# Autodesk Inventor assembly: I.A.B 2.1 Aracet
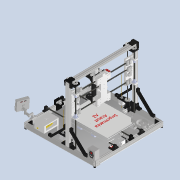
[picture p0: Inventor's stored thumbnail of the model, 180x180]
Saved by Autodesk Inventor 2020 (Build 240168000, 168)
## iProperties
Created: 2021-02-20
Part Number: I.A.B 2.1 Aracet
Document SubType Name: Assembly
Designer: Iulian Bors
Author: Iulian Bors
## Documents named in this file (72)
- Z:\I.A.B\Proiecte\0008 I.A.B 3D 2.1 Imprimanta aracet Metal\I.A.B 2.1 Aracet.iam
- Z:\I.A.B\Proiecte\0008 I.A.B 3D 2.1 Imprimanta aracet Metal\10 Mecanic\Foaie A3.ipt
- Z:\I.A.B\Proiecte\0008 I.A.B 3D 2.1 Imprimanta aracet Metal\10 Mecanic\0008-10-10 Injectomat Standard.iam
- Z:\I.A.B\Proiecte\0008 I.A.B 3D 2.1 Imprimanta aracet Metal\10 Mecanic\0008-10-006 suport injectomat.ipt
- Z:\I.A.B\Proiecte\0008 I.A.B 3D 2.1 Imprimanta aracet Metal\10 Mecanic\0008-10-1009 LM10uu.ipt
- Z:\I.A.B\Proiecte\0008 I.A.B 3D 2.1 Imprimanta aracet Metal\10 Mecanic\0008-10-007 Contra suport injectomat.ipt
- Z:\I.A.B\Proiecte\0008 I.A.B 3D 2.1 Imprimanta aracet Metal\10 Mecanic\0008-10-008 X Axis suport.ipt
- Z:\I.A.B\Proiecte\0008 I.A.B 3D 2.1 Imprimanta aracet Metal\10 Mecanic\0008-10-1001 NEMA17 - Motor de passo.ipt
- Z:\I.A.B\Proiecte\0008 I.A.B 3D 2.1 Imprimanta aracet Metal\10 Mecanic\0008-10-1011 GT2 Timing Pulley 20 Tooth.ipt
- Z:\I.A.B\Proiecte\0008 I.A.B 3D 2.1 Imprimanta aracet Metal\10 Mecanic\0008-10-009 X Axis suport.ipt
- Z:\I.A.B\Proiecte\0008 I.A.B 3D 2.1 Imprimanta aracet Metal\10 Mecanic\0008-10-010 Fixare AxaX.ipt
- Z:\I.A.B\Proiecte\0008 I.A.B 3D 2.1 Imprimanta aracet Metal\10 Mecanic\0008-10-011 Fixare AxaX Mijloc.ipt
- Z:\I.A.B\Proiecte\0008 I.A.B 3D 2.1 Imprimanta aracet Metal\10 Mecanic\0008-10-012 Intinzator X.ipt
- Z:\I.A.B\Proiecte\0008 I.A.B 3D 2.1 Imprimanta aracet Metal\10 Mecanic\0008-10-1012 16T W6 B3 Without T_Shrinkwrap_1.ipt
- Z:\I.A.B\Proiecte\0008 I.A.B 3D 2.1 Imprimanta aracet Metal\10 Mecanic\0008-10-1013 LMK 10 Bearing.ipt
- Z:\I.A.B\Proiecte\0008 I.A.B 3D 2.1 Imprimanta aracet Metal\10 Mecanic\0008-10-1010 Bara 10.ipt
- Z:\I.A.B\Proiecte\0008 I.A.B 3D 2.1 Imprimanta aracet Metal\10 Mecanic\0008-10-013 Supăort Piulita Axa Z.ipt
- Z:\I.A.B\Proiecte\0008 I.A.B 3D 2.1 Imprimanta aracet Metal\10 Mecanic\0008-10-1004 Piulita.ipt
- Z:\I.A.B\Proiecte\0008 I.A.B 3D 2.1 Imprimanta aracet Metal\10 Mecanic\0008-10-1014 T8 screw.ipt
- Z:\I.A.B\Proiecte\0008 I.A.B 3D 2.1 Imprimanta aracet Metal\10 Mecanic\0008-10-016 Suport Motor Z.ipt
- Z:\I.A.B\Proiecte\0008 I.A.B 3D 2.1 Imprimanta aracet Metal\10 Mecanic\0008-10-1005 ISO 1224-1 - 10 - 8 x 22 x 7.ipt
- Z:\I.A.B\Proiecte\0008 I.A.B 3D 2.1 Imprimanta aracet Metal\10 Mecanic\0008-10-015 roata condusa GT2.ipt
- Z:\I.A.B\Proiecte\0008 I.A.B 3D 2.1 Imprimanta aracet Metal\10 Mecanic\0008-10-1015 Synchronous Belt2.ipt
- Z:\I.A.B\Proiecte\0008 I.A.B 3D 2.1 Imprimanta aracet Metal\10 Mecanic\0008-10-017 Heated bed.ipt
- Z:\I.A.B\Proiecte\0008 I.A.B 3D 2.1 Imprimanta aracet Metal\10 Mecanic\0008-10-018 Suport Heated Bed.ipt
- Z:\I.A.B\Proiecte\0008 I.A.B 3D 2.1 Imprimanta aracet Metal\10 Mecanic\0008-10-1016 SC10UU.ipt
- Z:\I.A.B\Proiecte\0008 I.A.B 3D 2.1 Imprimanta aracet Metal\10 Mecanic\0008-10-1017 Bara 10.ipt
- Z:\I.A.B\Proiecte\0008 I.A.B 3D 2.1 Imprimanta aracet Metal\10 Mecanic\0008-10-019 Suport Axa Y.ipt
- Z:\I.A.B\Proiecte\0008 I.A.B 3D 2.1 Imprimanta aracet Metal\10 Mecanic\0008-10-1008 Bara 10_V1.ipt
- Z:\I.A.B\Proiecte\0008 I.A.B 3D 2.1 Imprimanta aracet Metal\10 Mecanic\0008-10-020 Suport Axa Y.ipt
- Z:\I.A.B\Proiecte\0008 I.A.B 3D 2.1 Imprimanta aracet Metal\10 Mecanic\0008-10-1018 V slot profiles.ipt
- Z:\I.A.B\Proiecte\0008 I.A.B 3D 2.1 Imprimanta aracet Metal\10 Mecanic\0008-10-1019 V slot profiles.ipt
- Z:\I.A.B\Proiecte\0008 I.A.B 3D 2.1 Imprimanta aracet Metal\10 Mecanic\0008-10-1020 V slot profiles.ipt
- Z:\I.A.B\Proiecte\0008 I.A.B 3D 2.1 Imprimanta aracet Metal\20 Electric\00008-20-1004 PowerSupplyLedMax500.ipt
- Z:\I.A.B\Proiecte\0008 I.A.B 3D 2.1 Imprimanta aracet Metal\10 Mecanic\0008-10-021 Suport Motor Z R.ipt
- Z:\I.A.B\Proiecte\0008 I.A.B 3D 2.1 Imprimanta aracet Metal\10 Mecanic\0008-10-1021  V slot profiles.ipt
- Z:\I.A.B\Proiecte\0008 I.A.B 3D 2.1 Imprimanta aracet Metal\10 Mecanic\0008-10-022 Tabla suport.ipt
- Z:\I.A.B\Proiecte\0008 I.A.B 3D 2.1 Imprimanta aracet Metal\10 Mecanic\0008-10-023 Suport L.ipt
- Z:\I.A.B\Proiecte\0008 I.A.B 3D 2.1 Imprimanta aracet Metal\10 Mecanic\0008-10-024 Ranforsare.ipt
- Z:\I.A.B\Proiecte\0008 I.A.B 3D 2.1 Imprimanta aracet Metal\10 Mecanic\0008-10-027 Cutie Arduino.ipt
- Z:\I.A.B\Proiecte\0008 I.A.B 3D 2.1 Imprimanta aracet Metal\10 Mecanic\0008-10-028 Cutie Elemente incalzire.ipt
- Z:\I.A.B\Proiecte\0008 I.A.B 3D 2.1 Imprimanta aracet Metal\20 Electric\0008-20-01 Assembly Arduino Mega RAMPS 1.4.iam
- Z:\I.A.B\Proiecte\0008 I.A.B 3D 2.1 Imprimanta aracet Metal\20 Electric\0008-20-1005 MOSFET_Step.ipt
- Z:\I.A.B\Proiecte\0008 I.A.B 3D 2.1 Imprimanta aracet Metal\10 Mecanic\0008-10-030 Suport L.ipt
- Z:\I.A.B\Proiecte\0008 I.A.B 3D 2.1 Imprimanta aracet Metal\10 Mecanic\0008-10-031 Suport L + placa.ipt
- Z:\I.A.B\Proiecte\0008 I.A.B 3D 2.1 Imprimanta aracet Metal\10 Mecanic\0008-10-1022 SHF10.ipt
- Z:\I.A.B\Proiecte\0008 I.A.B 3D 2.1 Imprimanta aracet Metal\10 Mecanic\0008-10-032 Suport cadru si axa Z.ipt
- Z:\I.A.B\Proiecte\0008 I.A.B 3D 2.1 Imprimanta aracet Metal\10 Mecanic\0008-10-033.ipt
- Z:\I.A.B\Proiecte\0008 I.A.B 3D 2.1 Imprimanta aracet Metal\10 Mecanic\0008-10-034 Suport_Rulment.ipt
- Z:\I.A.B\Proiecte\0008 I.A.B 3D 2.1 Imprimanta aracet Metal\10 Mecanic\0008-10-035.ipt
- Z:\I.A.B\Proiecte\0008 I.A.B 3D 2.1 Imprimanta aracet Metal\10 Mecanic\0008-10-037.ipt
- Z:\I.A.B\Proiecte\0008 I.A.B 3D 2.1 Imprimanta aracet Metal\10 Mecanic\0008-10-036.ipt
- Z:\I.A.B\Proiecte\0008 I.A.B 3D 2.1 Imprimanta aracet Metal\10 Mecanic\0008-10-11 ansamblu display.iam
- Z:\I.A.B\Proiecte\0008 I.A.B 3D 2.1 Imprimanta aracet Metal\10 Mecanic\0008-10-045.ipt
- Z:\I.A.B\Proiecte\0008 I.A.B 3D 2.1 Imprimanta aracet Metal\10 Mecanic\0008-10-044.ipt
- Z:\I.A.B\Proiecte\0008 I.A.B 3D 2.1 Imprimanta aracet Metal\10 Mecanic\0008-10-043.ipt
- Z:\I.A.B\Proiecte\0008 I.A.B 3D 2.1 Imprimanta aracet Metal\20 Electric\0008-20-1003 Switch.ipt
- Z:\I.A.B\Proiecte\0008 I.A.B 3D 2.1 Imprimanta aracet Metal\10 Mecanic\0008-10-046 Fixare axa si port cablu.ipt
- Z:\I.A.B\Proiecte\0008 I.A.B 3D 2.1 Imprimanta aracet Metal\10 Mecanic\0008-10-047 Suport Rulment Sc si curea.ipt
- Z:\I.A.B\Proiecte\0008 I.A.B 3D 2.1 Imprimanta aracet Metal\10 Mecanic\0008-10-048.ipt
- Z:\I.A.B\Proiecte\0008 I.A.B 3D 2.1 Imprimanta aracet Metal\10 Mecanic\0008-10-029 Capac Arduino.ipt
- Z:\I.A.B\Proiecte\0008 I.A.B 3D 2.1 Imprimanta aracet Metal\10 Mecanic\0008-10-049 Capac Mofset.ipt
- Z:\I.A.B\Proiecte\0008 I.A.B 3D 2.1 Imprimanta aracet Metal\10 Mecanic\Ansamblu nconector priza.iam
- Z:\I.A.B\Proiecte\0008 I.A.B 3D 2.1 Imprimanta aracet Metal\10 Mecanic\0008-10-056.ipt
- Z:\I.A.B\Proiecte\0008 I.A.B 3D 2.1 Imprimanta aracet Metal\10 Mecanic\0008-10-052 Suport Axa Y +Senzor.ipt
- Z:\I.A.B\Proiecte\0008 I.A.B 3D 2.1 Imprimanta aracet Metal\10 Mecanic\0008-10-026 Suport cutie.ipt
- Z:\I.A.B\Proiecte\0008 I.A.B 3D 2.1 Imprimanta aracet Metal\10 Mecanic\0008-10-053 picior.ipt
- Z:\I.A.B\Proiecte\0008 I.A.B 3D 2.1 Imprimanta aracet Metal\10 Mecanic\0008-10-054 Suport doking.ipt
- Z:\I.A.B\Proiecte\0008 I.A.B 3D 2.1 Imprimanta aracet Metal\10 Mecanic\0008-10-2016 DIN 315 - M4.ipt
- Z:\I.A.B\Proiecte\0008 I.A.B 3D 2.1 Imprimanta aracet Metal\10 Mecanic\0008-10-2017 DIN 7991 - M4x20.ipt
- Z:\I.A.B\Proiecte\0008 I.A.B 3D 2.1 Imprimanta aracet Metal\10 Mecanic\0008-10-055 Doking.ipt
- Z:\I.A.B\Proiecte\0008 I.A.B 3D 2.1 Imprimanta aracet Metal\10 Mecanic\0008-10-2000 DIN 6912 - M4 x 25.ipt
## Components (142 placed, 76 different names)
1. Foaie A3.ipt:1 — Mate:59, Flush:56, Flush:57, Angle:8, Mate:93
2. 0008-10-10 Injectomat Standard.iam:2 [sub-assembly] — Insert:10, Mate:64
3. 0008-10-006 suport injectomat.ipt:3 — Flush:3, Flush:4, Mate:8, Mate:9, Flush:5, Flush:6, Angle:2, Mate:17, Mate:23, Insert:10
4. 0008-10-1009 LM10uu.ipt:4 — Flush:1, Mate:5, Mate:8
5. 0008-10-1009 LM10uu.ipt:5 — Mate:5, Flush:121
6. 0008-10-1009 LM10uu.ipt:6 — Flush:4, Mate:6, Mate:9, Flush:1
7. 0008-10-1009 LM10uu.ipt:7 — Flush:3, Mate:6
8. 0008-10-007 Contra suport injectomat.ipt:8 — Flush:5, Flush:6, Mate:23, Mate:64, Flush:121, Flush:122, Mate:187, Flush:125, Flush:126
9. 0008-10-1008 Bara 10_V1.ipt:9
10. 0008-10-1008 Bara 10_V1.ipt:10 — Mate:188, Mate:189, Mate:191, Mate:192
11. 0008-10-009 X Axis suport.ipt:11 — Angle:2, Flush:10, Mate:21, Mate:22, Angle:3, Flush:26, Flush:27, Angle:4, Angle:5, Mate:26, Mate:27, Flush:32, Flush:34, Mate:38, Flush:36, Flush:37, Mate:163, Mate:164, Angle:28, Flush:127
12. 0008-10-008 X Axis suport.ipt:12 — Flush:10, Mate:21, Flush:31, Mate:30, Mate:31, Mate:33, Mate:34, Mate:35, Flush:89, Insert:21, Mate:172, Angle:25, Angle:29, Flush:128
13. 0008-10-1001 NEMA17 - Motor de passo.ipt:13 — Insert:1, Mate:22, Mate:26, Mate:27
14. 0008-10-1009 LM10uu.ipt:14 — Mate:17, Flush:122
15. 0008-10-1008 Bara 10_V1.ipt:15
16. 0008-10-1011 GT2 Timing Pulley 20 Tooth.ipt:16 — Insert:1, Flush:29, Flush:30, Angle:5
17. 0008-10-012 Intinzator X.ipt:17 — Flush:29, Insert:2, Flush:31
18. 0008-10-1012 16T W6 B3 Without T_Shrinkwrap_1.ipt:18 — Insert:2, Flush:30
19. 0008-10-1013 LMK 10 Bearing.ipt:19 — Mate:29, Angle:6, Mate:164
20. 0008-10-1013 LMK 10 Bearing.ipt:20 — Mate:33, Mate:34, Mate:35
21. 0008-10-1013 LMK 10 Bearing.ipt:21 — Mate:30, Mate:31, Mate:37, Angle:25
22. 0008-10-1013 LMK 10 Bearing.ipt:22 — Flush:32, Mate:29, Flush:34, Angle:6, Mate:36
23. 0008-10-010 Fixare AxaX.ipt:23 — Angle:3, Flush:26
24. 0008-10-1010 Bara 10.ipt:31 — Mate:36, Flush:35, Insert:15, Insert:16, Mate:163
25. 0008-10-1010 Bara 10.ipt:32 — Mate:37, Flush:35, Insert:17, Insert:18
26. 0008-10-013 Supăort Piulita Axa Z.ipt:33 — Mate:38, Flush:36, Mate:39, Mate:40, Flush:37, Flush:38
27. 0008-10-1004 Piulita.ipt:34 — Mate:39, Mate:40, Flush:38, Mate:44
28. 0008-10-013 Supăort Piulita Axa Z.ipt:35 — Insert:21, Mate:172, Mate:173, Mate:174
29. 0008-10-1004 Piulita.ipt:36 — Mate:45, Mate:173, Mate:174
30. 0008-10-1014 T8 screw.ipt:37 — Mate:44, Mate:47, Mate:50, Mate:168
31. 0008-10-1014 T8 screw.ipt:38 — Mate:45, Mate:57, Mate:58, Mate:82, Mate:113, Mate:171, Mate:176
32. 0008-10-016 Suport Motor Z.ipt:39 — Mate:47, Mate:48, Mate:49, Insert:6, Mate:101, Mate:103, Mate:104, Angle:14
33. 0008-10-1005 ISO 1224-1 - 10 - 8 x 22 x 7.ipt:40 — Insert:4, Insert:6
34. 0008-10-015 roata condusa GT2.ipt:41 — Insert:4, Mate:202
35. 0008-10-1001 NEMA17 - Motor de passo.ipt:42 — Insert:5, Mate:48, Mate:49
36. 0008-10-1011 GT2 Timing Pulley 20 Tooth.ipt:43 — Insert:5, Mate:51, Mate:52
37. 0008-10-1015 Synchronous Belt2.ipt:44 — Mate:50, Mate:51, Mate:52, Mate:202
38. 0008-10-016 Suport Motor Z.ipt:45 — Mate:82, Mate:87, Angle:15, Mate:107
39. 0008-10-1005 ISO 1224-1 - 10 - 8 x 22 x 7.ipt:46
40. 0008-10-015 roata condusa GT2.ipt:47 — Mate:57
41. 0008-10-1001 NEMA17 - Motor de passo.ipt:48 — Angle:16, Mate:113
42. 0008-10-1011 GT2 Timing Pulley 20 Tooth.ipt:49
43. 0008-10-1015 Synchronous Belt2.ipt:50 — Mate:58
44. 0008-10-017 Heated bed.ipt:51 — Mate:59, Flush:56, Flush:57, Mate:60, Mate:61, Mate:62
45. 0008-10-018 Suport Heated Bed.ipt:52 — Mate:60, Mate:61, Mate:62, Mate:65, Flush:59, Mate:66, Flush:61, Mate:68, Mate:69, Flush:64, Flush:65, Angle:9, Mate:73, Mate:74, Mate:78, Mate:197, Insert:32, Mate:210, Insert:33, Insert:36, Angle:32
46. 0008-10-1016 SC10UU.ipt:55 — Mate:69, Flush:63, Flush:64
47. 0008-10-1016 SC10UU.ipt:56 — Mate:66, Mate:67, Flush:60, Flush:63
48. 0008-10-1016 SC10UU.ipt:57 — Mate:68, Flush:62, Flush:65, Mate:70
49. 0008-10-1016 SC10UU.ipt:58 — Mate:65, Flush:59, Mate:67, Flush:60, Flush:61, Flush:62, Mate:77
50. 0008-10-1017 Bara 10.ipt:59 — Mate:70, Mate:71, Flush:66, Flush:67, Mate:72
51. 0008-10-019 Suport Axa Y.ipt:60 — Mate:71, Flush:66, Angle:9, Angle:10, Flush:70, Flush:71, Flush:73, Flush:74
52. 0008-10-019 Suport Axa Y.ipt:61 — Angle:10, Flush:67, Mate:72, Flush:75, Mate:208, Flush:138
53. 0008-10-1016 SC10UU:5 — Mate:73, Mate:74, Mate:78, Mate:79, Mate:198, Mate:199
54. 0008-10-1017 Bara 10:2 — Mate:77, Flush:72
55. 0008-10-020 Suport Axa Y:4 — Flush:70, Flush:71, Mate:135
56. 0008-10-020 Suport Axa Y:6 — Angle:12
57. 0008-10-1017 Bara 10:3 — Mate:79, Flush:72, Mate:80, Mate:81
58. 0008-10-019 Suport Axa Y:2 — Mate:80, Flush:73, Flush:74, Mate:83, Flush:77, Angle:27, Mate:182
59. 0008-10-019 Suport Axa Y:1 — Mate:81, Flush:75, Angle:12
60. 0008-10-1018 V slot profiles:1 — Mate:83, Flush:77, Flush:78, Mate:85, Flush:79, Flush:80, Mate:86, Flush:81, Mate:93, Mate:109, Flush:101, Mate:112, Mate:114, Angle:17, Mate:136, Flush:110, Mate:183, Mate:186, Flush:123, Flush:124
61. 0008-10-1019 V slot profiles:1 — Flush:78, Mate:85, Flush:79, Mate:100, Flush:96, Mate:101, Angle:14, Mate:105, Flush:102, Mate:111, Flush:104, Mate:122, Mate:123, Flush:105, Mate:125, Flush:106, Mate:129, Flush:108, Mate:152, Mate:156, Mate:157, Angle:20, Mate:205, Flush:133
62. 0008-10-1019 V slot profiles:2 — Flush:80, Mate:86, Flush:81, Mate:87, Flush:82, Flush:85, Mate:90, Flush:94, Mate:99, Flush:95, Angle:15, Mate:106, Flush:100, Angle:16, Mate:116, Mate:119, Mate:127, Mate:132, Mate:141, Flush:113, Mate:143, Flush:114, Mate:146, Mate:149, Angle:19
63. 0008-10-1018 V slot profiles:2 — Flush:82, Flush:85, Mate:90, Mate:97, Flush:99, Mate:108, Flush:103, Mate:118, Mate:121, Mate:200, Flush:131, Flush:134
64. 0008-10-1018 V slot profiles:3 — Flush:97, Flush:98, Mate:110, Mate:161, Angle:22, Mate:165, Flush:116, Angle:24, Mate:170, Mate:177
65. 0008-10-1020 V slot profiles:2 — Flush:89, Flush:91, Mate:99, Flush:95, Flush:97, Flush:98, Mate:128, Flush:107, Mate:131, Flush:109, Mate:142, Mate:144, Mate:169, Flush:117, Flush:118, Mate:178
66. 0008-10-1020 V slot profiles:3 — Flush:91, Mate:100, Flush:96, Flush:103, Mate:110, Mate:124, Mate:126, Mate:158, Mate:159, Mate:162, Flush:115, Mate:166, Mate:207, Flush:137
67. 0008-10-1001 NEMA17 - Motor de passo:4 — Mate:97, Flush:99, Mate:201
68. 0008-10-1011 GT2 Timing Pulley 20 Tooth:4 — Flush:120
69. 00008-20-1004 PowerSupplyLedMax500:1 — Flush:94, Mate:108, Flush:130, Mate:195, Mate:196
70. 0008-10-1021  V slot profiles:1 — Mate:103, Mate:104, Mate:105, Mate:153, Mate:155, Flush:132
71. 0008-10-1021  V slot profiles:2 — Mate:106, Mate:107, Flush:100, Mate:147, Mate:150, Flush:132
72. 0008-10-022 Tabla suport:1 — Mate:109, Flush:101, Flush:102, Mate:115, Mate:117, Mate:120, Mate:130, Mate:145, Mate:148, Mate:151, Mate:154, Mate:160, Mate:180, Mate:194, Insert:28, Insert:29, Insert:30, Insert:31
73. 0008-10-023 Suport L:1 — Mate:111, Flush:104, Mate:112
74. 0008-10-023 Suport L:2 — Mate:120, Mate:121, Mate:122
75. 0008-10-023 Suport L:3 — Mate:117, Mate:118, Mate:119, Mate:196
76. 0008-10-023 Suport L:4 — Mate:114, Mate:115, Mate:116
77. 0008-10-024 Ranforsare:1 — Mate:123, Flush:105, Mate:124
78. 0008-10-024 Ranforsare:2 — Mate:127, Mate:128, Flush:107
79. 0008-10-024 Ranforsare:3 — Mate:125, Mate:126, Flush:106
80. 0008-10-027 Cutie Arduino:1 — Mate:129, Flush:108, Insert:12, Angle:18, Flush:110, Insert:26, Angle:30, Insert:27, Mate:209
81. 0008-10-028 Cutie Elemente incalzire:1 — Mate:130, Angle:17, Insert:13, Mate:133, Insert:14, Mate:134, Mate:135, Mate:136, Mate:203, Mate:204, Angle:31
82. 0008-10-024 Ranforsare:4 — Mate:131, Flush:109, Mate:132
83. 0008-20-01 Assembly Arduino Mega RAMPS 1.4:1 [sub-assembly] — Insert:12, Angle:18
84. 0008-20-1005 MOSFET_Step:1 — Insert:13, Mate:133
85. 0008-20-1005 MOSFET_Step:2 — Insert:14, Mate:134
86. 0008-10-031 Suport L + placa:1 — Mate:143, Mate:144, Flush:114
87. 0008-10-030 Suport L:4 — Mate:141, Mate:142, Flush:113
88. 0008-10-030 Suport L:5 — Mate:145, Mate:146, Mate:147
89. 0008-10-030 Suport L:6 — Mate:148, Mate:149, Mate:150
90. 0008-10-031 Suport L + placa:2 — Mate:157, Mate:158, Mate:159
91. 0008-10-030 Suport L:7 — Mate:151, Mate:152, Mate:153
92. 0008-10-030 Suport L:8 — Mate:154, Mate:155, Mate:156
93. 0008-10-1022 SHF10:1 — Insert:16, Mate:160, Angle:20
94. 0008-10-1022 SHF10:2 — Insert:18, Angle:19
95. 0008-10-1022 SHF10:3 — Insert:17, Angle:22
96. 0008-10-1022 SHF10:4 — Insert:15, Angle:23
97. 0008-10-032 Suport cadru si axa Z:1 — Mate:161, Mate:162, Flush:115
98. 0008-10-033:1 — Mate:165, Flush:116, Mate:166, Angle:23, Mate:167
99. 0008-10-034 Suport_Rulment:1 — Mate:167, Angle:24
100. ISO 1224-1 (Metric) 10 - 8 x 16 x 7:3 — Mate:168
101. 0008-10-035:1 — Mate:169, Flush:117, Mate:170, Mate:171, Mate:175
102. 0008-10-034 Suport_Rulment:2 — Mate:175
103. ISO 1224-1 (Metric) 10 - 8 x 16 x 7:4 — Mate:176
104. 0008-10-032 Suport cadru si axa Z:2 — Mate:177, Flush:118, Mate:178
105. 0008-10-037:1 — Mate:180, Mate:181, Mate:182, Mate:183, Mate:184
106. 0008-10-036:1 — Insert:22, Angle:27, Mate:181, Mate:184
107. 0008-10-1012 16T W6 B3 Without T_Shrinkwrap_1:2 — Insert:22, Flush:120
108. 0008-10-11 ansamblu display:1 [sub-assembly] — Insert:23, Mate:185
109. 0008-10-045:1 — Insert:23, Mate:185, Insert:24
110. 0008-10-044:1 — Insert:24, Insert:25
111. 0008-10-043:1 — Mate:186, Flush:123, Insert:25, Flush:124
112. 0008-20-1003 Switch:1 — Mate:187, Flush:125, Flush:126
113. 0008-10-010 Fixare AxaX:2 — Mate:188, Angle:28, Flush:127, Mate:190
114. 0008-10-010 Fixare AxaX:4 — Mate:189, Mate:190
115. 00008-20-1004 PowerSupplyLedMax500:2 — Mate:194, Flush:130, Mate:195
116. 0008-10-047 Suport Rulment Sc si curea:1 — Mate:197, Mate:198, Mate:199
117. 0008-10-048:1 — Mate:200, Mate:201, Flush:131
118. 0008-10-029 Capac Arduino:1 — Insert:26, Angle:30
119. 0008-10-049 Capac Mofset:1 — Mate:203, Mate:204, Angle:31
120. Ansamblu nconector priza:1 [sub-assembly] — Mate:205, Flush:133, Flush:134
121. 0008-20-1003 Switch:2 — Mate:206, Flush:135, Flush:136
122. 0008-10-056:1 — Mate:206, Flush:135, Flush:136, Mate:207, Flush:137
123. 0008-20-1003 Switch:3 — Mate:208, Flush:138
124. 0008-10-026 Suport cutie:1 — Insert:27, Mate:209
125. 0008-10-053 picior:1 — Insert:28
126. 0008-10-053 picior:3 — Insert:31
127. 0008-10-053 picior:4 — Insert:30
128. 0008-10-053 picior:5 — Insert:29
129. 0008-10-054 Suport doking:1 — Insert:32, Mate:210, Flush:139, Mate:211, Mate:212, Insert:39
130. DIN 315 M4:1 — Insert:34
131. DIN 7991 M4x20:1 — Insert:33, Insert:34
132. DIN 315 M4:2
133. DIN 7991 M4x20:2 — Insert:36
134. 0008-10-055 Doking:1 — Flush:139, Angle:32, Mate:211, Mate:212
135. DIN 315 M4:3 — Insert:40
136. DIN 6912 M4 x 25:1 — Insert:39, Insert:40
137. 0008-10-011 Fixare AxaX Mijloc.ipt:53 — Flush:27, Angle:4
138. 0008-10-011 Fixare AxaX Mijloc.ipt:54
139. 0008-10-010 Fixare AxaX:5 — Mate:191, Angle:29, Flush:128, Flush:129, Mate:193
140. 0008-10-010 Fixare AxaX:3 — Mate:192, Flush:129, Mate:193
141. 0008-10-010 Fixare AxaX:6
142. 0008-10-010 Fixare AxaX:7
## Component patterns: (2 elements, first: 0008-10-011 Fixare AxaX Mijloc.ipt:53), (2 elements, first: 0008-10-010 Fixare AxaX:5 + 0008-10-010 Fixare AxaX:3)
## Relationships (336: Mate 179, Flush 92, Insert 37, Angle 27, Tangent 1)
- Flush:1 (20 mm): 0008-10-1009 LM10uu.ipt:4 ↔ 0008-10-1009 LM10uu.ipt:6
- Mate:5: 0008-10-1009 LM10uu.ipt:4 ↔ 0008-10-1009 LM10uu.ipt:5
- Flush:3 (20 mm): 0008-10-006 suport injectomat.ipt:3 ↔ 0008-10-1009 LM10uu.ipt:7
- Flush:4 (20 mm): 0008-10-006 suport injectomat.ipt:3 ↔ 0008-10-1009 LM10uu.ipt:6
- Mate:6: 0008-10-1009 LM10uu.ipt:6 ↔ 0008-10-1009 LM10uu.ipt:7
- Mate:8: 0008-10-006 suport injectomat.ipt:3 ↔ 0008-10-1009 LM10uu.ipt:4
- Mate:9: 0008-10-006 suport injectomat.ipt:3 ↔ 0008-10-1009 LM10uu.ipt:6
- Flush:5: 0008-10-006 suport injectomat.ipt:3 ↔ 0008-10-007 Contra suport injectomat.ipt:8
- Flush:6: 0008-10-006 suport injectomat.ipt:3 ↔ 0008-10-007 Contra suport injectomat.ipt:8
- [Mate]: 0008-10-1009 LM10uu.ipt:5 ↔ 0008-10-1008 Bara 10_V1.ipt:9
- [Mate]: 0008-10-1009 LM10uu.ipt:7 ↔ 0008-10-1008 Bara 10_V1.ipt:10
- [Flush]: 0008-10-1008 Bara 10_V1.ipt:9 ↔ 0008-10-1008 Bara 10_V1.ipt:10
- [Tangent] (-3 mm): 0008-10-1008 Bara 10_V1.ipt:9 ↔ 0008-10-009 X Axis suport.ipt:11
- Angle:2 (0 deg): 0008-10-006 suport injectomat.ipt:3 ↔ 0008-10-009 X Axis suport.ipt:11
- [Flush] (-30 mm): 0008-10-1008 Bara 10_V1.ipt:9 ↔ 0008-10-009 X Axis suport.ipt:11
- Flush:10: 0008-10-009 X Axis suport.ipt:11 ↔ 0008-10-008 X Axis suport.ipt:12
- [Flush] (-30 mm): 0008-10-1008 Bara 10_V1.ipt:9 ↔ 0008-10-008 X Axis suport.ipt:12
- Mate:21: 0008-10-009 X Axis suport.ipt:11 ↔ 0008-10-008 X Axis suport.ipt:12
- [Mate]: Foaie A3.ipt:1 ↔ 0008-10-1008 Bara 10_V1.ipt:9
- Mate:17: 0008-10-006 suport injectomat.ipt:3 ↔ 0008-10-1009 LM10uu.ipt:14
- Insert:1: 0008-10-1001 NEMA17 - Motor de passo.ipt:13 ↔ 0008-10-1011 GT2 Timing Pulley 20 Tooth.ipt:16
- Mate:22 (-10 mm): 0008-10-009 X Axis suport.ipt:11 ↔ 0008-10-1001 NEMA17 - Motor de passo.ipt:13
- Mate:23 (2 mm): 0008-10-006 suport injectomat.ipt:3 ↔ 0008-10-007 Contra suport injectomat.ipt:8
- [Flush]: 0008-10-1008 Bara 10_V1.ipt:9 ↔ 0008-10-1008 Bara 10_V1.ipt:15
- [Mate]: 0008-10-1009 LM10uu.ipt:14 ↔ 0008-10-1008 Bara 10_V1.ipt:15
- [Mate]: 0008-10-1008 Bara 10_V1.ipt:9 ↔ 0008-10-010 Fixare AxaX.ipt:23
- Angle:3 (0 deg): 0008-10-009 X Axis suport.ipt:11 ↔ 0008-10-010 Fixare AxaX.ipt:23
- Flush:26 (35 mm): 0008-10-009 X Axis suport.ipt:11 ↔ 0008-10-010 Fixare AxaX.ipt:23
- [Mate]: 0008-10-1008 Bara 10_V1.ipt:15 ↔ 0008-10-011 Fixare AxaX Mijloc.ipt:53
- Flush:27 (30 mm): 0008-10-009 X Axis suport.ipt:11 ↔ 0008-10-011 Fixare AxaX Mijloc.ipt:53
- Angle:4 (0 deg): 0008-10-009 X Axis suport.ipt:11 ↔ 0008-10-011 Fixare AxaX Mijloc.ipt:53
- Flush:29: 0008-10-1011 GT2 Timing Pulley 20 Tooth.ipt:16 ↔ 0008-10-012 Intinzator X.ipt:17
- Insert:2 (0.25 mm): 0008-10-012 Intinzator X.ipt:17 ↔ 0008-10-1012 16T W6 B3 Without T_Shrinkwrap_1.ipt:18
- Flush:30: 0008-10-1011 GT2 Timing Pulley 20 Tooth.ipt:16 ↔ 0008-10-1012 16T W6 B3 Without T_Shrinkwrap_1.ipt:18
- Flush:31: 0008-10-008 X Axis suport.ipt:12 ↔ 0008-10-012 Intinzator X.ipt:17
- Angle:5 (0 deg): 0008-10-009 X Axis suport.ipt:11 ↔ 0008-10-1011 GT2 Timing Pulley 20 Tooth.ipt:16
- Mate:26 (1 mm): 0008-10-009 X Axis suport.ipt:11 ↔ 0008-10-1001 NEMA17 - Motor de passo.ipt:13
- Mate:27 (1 mm): 0008-10-009 X Axis suport.ipt:11 ↔ 0008-10-1001 NEMA17 - Motor de passo.ipt:13
- Flush:32 (15 mm): 0008-10-009 X Axis suport.ipt:11 ↔ 0008-10-1013 LMK 10 Bearing.ipt:22
- Mate:29: 0008-10-1013 LMK 10 Bearing.ipt:19 ↔ 0008-10-1013 LMK 10 Bearing.ipt:22
- Flush:34: 0008-10-009 X Axis suport.ipt:11 ↔ 0008-10-1013 LMK 10 Bearing.ipt:22
- Angle:6 (0 deg): 0008-10-1013 LMK 10 Bearing.ipt:19 ↔ 0008-10-1013 LMK 10 Bearing.ipt:22
- Mate:30: 0008-10-008 X Axis suport.ipt:12 ↔ 0008-10-1013 LMK 10 Bearing.ipt:21
- Mate:31: 0008-10-008 X Axis suport.ipt:12 ↔ 0008-10-1013 LMK 10 Bearing.ipt:21
- Mate:33: 0008-10-008 X Axis suport.ipt:12 ↔ 0008-10-1013 LMK 10 Bearing.ipt:20
- Mate:34: 0008-10-008 X Axis suport.ipt:12 ↔ 0008-10-1013 LMK 10 Bearing.ipt:20
- Mate:35: 0008-10-008 X Axis suport.ipt:12 ↔ 0008-10-1013 LMK 10 Bearing.ipt:20
- Mate:36: 0008-10-1013 LMK 10 Bearing.ipt:22 ↔ 0008-10-1010 Bara 10.ipt:31
- Mate:37: 0008-10-1013 LMK 10 Bearing.ipt:21 ↔ 0008-10-1010 Bara 10.ipt:32
- Flush:35: 0008-10-1010 Bara 10.ipt:31 ↔ 0008-10-1010 Bara 10.ipt:32
- Mate:38: 0008-10-009 X Axis suport.ipt:11 ↔ 0008-10-013 Supăort Piulita Axa Z.ipt:33
- Flush:36: 0008-10-009 X Axis suport.ipt:11 ↔ 0008-10-013 Supăort Piulita Axa Z.ipt:33
- Mate:39: 0008-10-013 Supăort Piulita Axa Z.ipt:33 ↔ 0008-10-1004 Piulita.ipt:34
- Mate:40 (-12 mm): 0008-10-013 Supăort Piulita Axa Z.ipt:33 ↔ 0008-10-1004 Piulita.ipt:34
- Flush:37 (80 mm): 0008-10-009 X Axis suport.ipt:11 ↔ 0008-10-013 Supăort Piulita Axa Z.ipt:33
- Flush:38 (15 mm): 0008-10-013 Supăort Piulita Axa Z.ipt:33 ↔ 0008-10-1004 Piulita.ipt:34
- Mate:44: 0008-10-1004 Piulita.ipt:34 ↔ 0008-10-1014 T8 screw.ipt:37
- Mate:45: 0008-10-1004 Piulita.ipt:36 ↔ 0008-10-1014 T8 screw.ipt:38
- Insert:4: 0008-10-1005 ISO 1224-1 - 10 - 8 x 22 x 7.ipt:40 ↔ 0008-10-015 roata condusa GT2.ipt:41
- Mate:47 (1 mm): 0008-10-1014 T8 screw.ipt:37 ↔ 0008-10-016 Suport Motor Z.ipt:39
- Insert:5: 0008-10-1001 NEMA17 - Motor de passo.ipt:42 ↔ 0008-10-1011 GT2 Timing Pulley 20 Tooth.ipt:43
- Mate:48: 0008-10-016 Suport Motor Z.ipt:39 ↔ 0008-10-1001 NEMA17 - Motor de passo.ipt:42
- Mate:49: 0008-10-016 Suport Motor Z.ipt:39 ↔ 0008-10-1001 NEMA17 - Motor de passo.ipt:42
- Mate:50: 0008-10-1014 T8 screw.ipt:37 ↔ 0008-10-1015 Synchronous Belt2.ipt:44
- Mate:51: 0008-10-1011 GT2 Timing Pulley 20 Tooth.ipt:43 ↔ 0008-10-1015 Synchronous Belt2.ipt:44
- Mate:52 (1.5 mm): 0008-10-1011 GT2 Timing Pulley 20 Tooth.ipt:43 ↔ 0008-10-1015 Synchronous Belt2.ipt:44
- Insert:6: 0008-10-016 Suport Motor Z.ipt:39 ↔ 0008-10-1005 ISO 1224-1 - 10 - 8 x 22 x 7.ipt:40
- [Insert]: 0008-10-1005 ISO 1224-1 - 10 - 8 x 22 x 7.ipt:46 ↔ 0008-10-015 roata condusa GT2.ipt:47
- [Insert]: 0008-10-1001 NEMA17 - Motor de passo.ipt:48 ↔ 0008-10-1011 GT2 Timing Pulley 20 Tooth.ipt:49
- [Mate]: 0008-10-016 Suport Motor Z.ipt:45 ↔ 0008-10-1001 NEMA17 - Motor de passo.ipt:48
- [Mate]: 0008-10-1011 GT2 Timing Pulley 20 Tooth.ipt:49 ↔ 0008-10-1015 Synchronous Belt2.ipt:50
- [Mate] (1.5 mm): 0008-10-1011 GT2 Timing Pulley 20 Tooth.ipt:49 ↔ 0008-10-1015 Synchronous Belt2.ipt:50
- [Insert]: 0008-10-016 Suport Motor Z.ipt:45 ↔ 0008-10-1005 ISO 1224-1 - 10 - 8 x 22 x 7.ipt:46
- Mate:57: 0008-10-1014 T8 screw.ipt:38 ↔ 0008-10-015 roata condusa GT2.ipt:47
- Mate:58: 0008-10-1014 T8 screw.ipt:38 ↔ 0008-10-1015 Synchronous Belt2.ipt:50
- Mate:59: Foaie A3.ipt:1 ↔ 0008-10-017 Heated bed.ipt:51
- Flush:56 (-10 mm): Foaie A3.ipt:1 ↔ 0008-10-017 Heated bed.ipt:51
- Flush:57 (-10 mm): Foaie A3.ipt:1 ↔ 0008-10-017 Heated bed.ipt:51
- Mate:60 (25 mm): 0008-10-017 Heated bed.ipt:51 ↔ 0008-10-018 Suport Heated Bed.ipt:52
- Mate:61: 0008-10-017 Heated bed.ipt:51 ↔ 0008-10-018 Suport Heated Bed.ipt:52
- Mate:62: 0008-10-017 Heated bed.ipt:51 ↔ 0008-10-018 Suport Heated Bed.ipt:52
- Angle:8 (0 deg): Foaie A3.ipt:1
- [Mate]: 0008-10-1008 Bara 10_V1.ipt:9 ↔ 0008-10-009 X Axis suport.ipt:11
- Insert:10: 0008-10-10 Injectomat Standard.iam:2 ↔ 0008-10-006 suport injectomat.ipt:3
- Mate:64: 0008-10-10 Injectomat Standard.iam:2 ↔ 0008-10-007 Contra suport injectomat.ipt:8
- Mate:65: 0008-10-018 Suport Heated Bed.ipt:52 ↔ 0008-10-1016 SC10UU.ipt:58
- Flush:59 (5 mm): 0008-10-018 Suport Heated Bed.ipt:52 ↔ 0008-10-1016 SC10UU.ipt:58
- Mate:66: 0008-10-018 Suport Heated Bed.ipt:52 ↔ 0008-10-1016 SC10UU.ipt:56
- Mate:67 (100 mm): 0008-10-1016 SC10UU.ipt:56 ↔ 0008-10-1016 SC10UU.ipt:58
- Flush:60: 0008-10-1016 SC10UU.ipt:56 ↔ 0008-10-1016 SC10UU.ipt:58
- Flush:61 (135 mm): 0008-10-018 Suport Heated Bed.ipt:52 ↔ 0008-10-1016 SC10UU.ipt:58
- Mate:68: 0008-10-018 Suport Heated Bed.ipt:52 ↔ 0008-10-1016 SC10UU.ipt:57
- Flush:62: 0008-10-1016 SC10UU.ipt:57 ↔ 0008-10-1016 SC10UU.ipt:58
- Mate:69: 0008-10-018 Suport Heated Bed.ipt:52 ↔ 0008-10-1016 SC10UU.ipt:55
- Flush:63: 0008-10-1016 SC10UU.ipt:55 ↔ 0008-10-1016 SC10UU.ipt:56
- Flush:64 (5 mm): 0008-10-018 Suport Heated Bed.ipt:52 ↔ 0008-10-1016 SC10UU.ipt:55
- Flush:65 (5 mm): 0008-10-018 Suport Heated Bed.ipt:52 ↔ 0008-10-1016 SC10UU.ipt:57
- Mate:70: 0008-10-1016 SC10UU.ipt:57 ↔ 0008-10-1017 Bara 10.ipt:59
- Mate:71: 0008-10-1017 Bara 10.ipt:59 ↔ 0008-10-019 Suport Axa Y.ipt:60
- Flush:66: 0008-10-1017 Bara 10.ipt:59 ↔ 0008-10-019 Suport Axa Y.ipt:60
- Angle:9 (0 deg): 0008-10-018 Suport Heated Bed.ipt:52 ↔ 0008-10-019 Suport Axa Y.ipt:60
- Angle:10 (0 deg): 0008-10-019 Suport Axa Y.ipt:60 ↔ 0008-10-019 Suport Axa Y.ipt:61
- Flush:67: 0008-10-1017 Bara 10.ipt:59 ↔ 0008-10-019 Suport Axa Y.ipt:61
- Mate:72: 0008-10-1017 Bara 10.ipt:59 ↔ 0008-10-019 Suport Axa Y.ipt:61
- Mate:73 (5 mm): 0008-10-018 Suport Heated Bed.ipt:52 ↔ 0008-10-1016 SC10UU:5
- Mate:74 (30 mm): 0008-10-018 Suport Heated Bed.ipt:52 ↔ 0008-10-1016 SC10UU:5
- [Mate]: 0008-10-1017 Bara 10:2 ↔ 0008-10-020 Suport Axa Y:4
- [Flush]: 0008-10-1017 Bara 10:2 ↔ 0008-10-020 Suport Axa Y:4
- [Angle] (0 deg): 0008-10-020 Suport Axa Y:4 ↔ 0008-10-020 Suport Axa Y:6
- [Flush]: 0008-10-1017 Bara 10:2 ↔ 0008-10-020 Suport Axa Y:6
- [Mate]: 0008-10-1017 Bara 10:2 ↔ 0008-10-020 Suport Axa Y:6
- Mate:77: 0008-10-1016 SC10UU.ipt:58 ↔ 0008-10-1017 Bara 10:2
- Mate:78 (-17.5 mm): 0008-10-018 Suport Heated Bed.ipt:52 ↔ 0008-10-1016 SC10UU:5
- Flush:70: 0008-10-019 Suport Axa Y.ipt:60 ↔ 0008-10-020 Suport Axa Y:4
- Flush:71: 0008-10-019 Suport Axa Y.ipt:60 ↔ 0008-10-020 Suport Axa Y:4
- Mate:79: 0008-10-1016 SC10UU:5 ↔ 0008-10-1017 Bara 10:3
- Flush:72: 0008-10-1017 Bara 10:2 ↔ 0008-10-1017 Bara 10:3
- Mate:80: 0008-10-1017 Bara 10:3 ↔ 0008-10-019 Suport Axa Y:2
- Flush:73: 0008-10-019 Suport Axa Y.ipt:60 ↔ 0008-10-019 Suport Axa Y:2
- Flush:74: 0008-10-019 Suport Axa Y.ipt:60 ↔ 0008-10-019 Suport Axa Y:2
- Mate:81: 0008-10-1017 Bara 10:3 ↔ 0008-10-019 Suport Axa Y:1
- Flush:75: 0008-10-019 Suport Axa Y.ipt:61 ↔ 0008-10-019 Suport Axa Y:1
- Mate:82 (1 mm): 0008-10-1014 T8 screw.ipt:38 ↔ 0008-10-016 Suport Motor Z.ipt:45
- Mate:83: 0008-10-019 Suport Axa Y:2 ↔ 0008-10-1018 V slot profiles:1
- Flush:77: 0008-10-019 Suport Axa Y:2 ↔ 0008-10-1018 V slot profiles:1
- Flush:78: 0008-10-1018 V slot profiles:1 ↔ 0008-10-1019 V slot profiles:1
- Mate:85: 0008-10-1018 V slot profiles:1 ↔ 0008-10-1019 V slot profiles:1
- Flush:79: 0008-10-1018 V slot profiles:1 ↔ 0008-10-1019 V slot profiles:1
- Flush:80: 0008-10-1018 V slot profiles:1 ↔ 0008-10-1019 V slot profiles:2
- Mate:86: 0008-10-1018 V slot profiles:1 ↔ 0008-10-1019 V slot profiles:2
- Flush:81: 0008-10-1018 V slot profiles:1 ↔ 0008-10-1019 V slot profiles:2
- Mate:87: 0008-10-016 Suport Motor Z.ipt:45 ↔ 0008-10-1019 V slot profiles:2
- Flush:82: 0008-10-1019 V slot profiles:2 ↔ 0008-10-1018 V slot profiles:2
- Angle:12 (0 deg): 0008-10-020 Suport Axa Y:6 ↔ 0008-10-019 Suport Axa Y:1
- Flush:85: 0008-10-1019 V slot profiles:2 ↔ 0008-10-1018 V slot profiles:2
- Mate:90: 0008-10-1019 V slot profiles:2 ↔ 0008-10-1018 V slot profiles:2
- Mate:93: Foaie A3.ipt:1 ↔ 0008-10-1018 V slot profiles:1
- Flush:89 (-12.5 mm): 0008-10-008 X Axis suport.ipt:12 ↔ 0008-10-1020 V slot profiles:2
- Flush:91: 0008-10-1020 V slot profiles:2 ↔ 0008-10-1020 V slot profiles:3
- [Insert]: 0008-10-1001 NEMA17 - Motor de passo:4 ↔ 0008-10-1011 GT2 Timing Pulley 20 Tooth:4
- Mate:97: 0008-10-1018 V slot profiles:2 ↔ 0008-10-1001 NEMA17 - Motor de passo:4
- Flush:94: 0008-10-1019 V slot profiles:2 ↔ 00008-20-1004 PowerSupplyLedMax500:1
- Mate:99: 0008-10-1019 V slot profiles:2 ↔ 0008-10-1020 V slot profiles:2
- Flush:95: 0008-10-1019 V slot profiles:2 ↔ 0008-10-1020 V slot profiles:2
- Mate:100: 0008-10-1019 V slot profiles:1 ↔ 0008-10-1020 V slot profiles:3
- Flush:96: 0008-10-1019 V slot profiles:1 ↔ 0008-10-1020 V slot profiles:3
- Flush:97: 0008-10-1018 V slot profiles:3 ↔ 0008-10-1020 V slot profiles:2
- Flush:98: 0008-10-1018 V slot profiles:3 ↔ 0008-10-1020 V slot profiles:2
- Flush:99: 0008-10-1018 V slot profiles:2 ↔ 0008-10-1001 NEMA17 - Motor de passo:4
- Mate:101: 0008-10-016 Suport Motor Z.ipt:39 ↔ 0008-10-1019 V slot profiles:1
- Mate:103: 0008-10-016 Suport Motor Z.ipt:39 ↔ 0008-10-1021  V slot profiles:1
- Mate:104: 0008-10-016 Suport Motor Z.ipt:39 ↔ 0008-10-1021  V slot profiles:1
- Angle:14 (0 deg): 0008-10-016 Suport Motor Z.ipt:39 ↔ 0008-10-1019 V slot profiles:1
- Mate:105: 0008-10-1019 V slot profiles:1 ↔ 0008-10-1021  V slot profiles:1
- Angle:15 (0 deg): 0008-10-016 Suport Motor Z.ipt:45 ↔ 0008-10-1019 V slot profiles:2
- Mate:106: 0008-10-1019 V slot profiles:2 ↔ 0008-10-1021  V slot profiles:2
- Mate:107: 0008-10-016 Suport Motor Z.ipt:45 ↔ 0008-10-1021  V slot profiles:2
- Flush:100: 0008-10-1019 V slot profiles:2 ↔ 0008-10-1021  V slot profiles:2
- Mate:108: 0008-10-1018 V slot profiles:2 ↔ 00008-20-1004 PowerSupplyLedMax500:1
- Mate:109: 0008-10-1018 V slot profiles:1 ↔ 0008-10-022 Tabla suport:1
- Flush:101: 0008-10-1018 V slot profiles:1 ↔ 0008-10-022 Tabla suport:1
- Flush:102: 0008-10-1019 V slot profiles:1 ↔ 0008-10-022 Tabla suport:1
- Flush:103 (250.528 mm): 0008-10-1018 V slot profiles:2 ↔ 0008-10-1020 V slot profiles:3
- Mate:110: 0008-10-1018 V slot profiles:3 ↔ 0008-10-1020 V slot profiles:3
- Mate:111: 0008-10-1019 V slot profiles:1 ↔ 0008-10-023 Suport L:1
- Flush:104: 0008-10-1019 V slot profiles:1 ↔ 0008-10-023 Suport L:1
- Mate:112: 0008-10-1018 V slot profiles:1 ↔ 0008-10-023 Suport L:1
- Angle:16 (0 deg): 0008-10-1001 NEMA17 - Motor de passo.ipt:48 ↔ 0008-10-1019 V slot profiles:2
- Mate:113: 0008-10-1014 T8 screw.ipt:38 ↔ 0008-10-1001 NEMA17 - Motor de passo.ipt:48
- Mate:114: 0008-10-1018 V slot profiles:1 ↔ 0008-10-023 Suport L:4
- Mate:115: 0008-10-022 Tabla suport:1 ↔ 0008-10-023 Suport L:4
- Mate:116: 0008-10-1019 V slot profiles:2 ↔ 0008-10-023 Suport L:4
- Mate:117: 0008-10-022 Tabla suport:1 ↔ 0008-10-023 Suport L:3
- Mate:118: 0008-10-1018 V slot profiles:2 ↔ 0008-10-023 Suport L:3
- Mate:119: 0008-10-1019 V slot profiles:2 ↔ 0008-10-023 Suport L:3
- Mate:120: 0008-10-022 Tabla suport:1 ↔ 0008-10-023 Suport L:2
- Mate:121: 0008-10-1018 V slot profiles:2 ↔ 0008-10-023 Suport L:2
- Mate:122: 0008-10-1019 V slot profiles:1 ↔ 0008-10-023 Suport L:2
- Mate:123: 0008-10-1019 V slot profiles:1 ↔ 0008-10-024 Ranforsare:1
- Flush:105: 0008-10-1019 V slot profiles:1 ↔ 0008-10-024 Ranforsare:1
- Mate:124: 0008-10-1020 V slot profiles:3 ↔ 0008-10-024 Ranforsare:1
- Mate:125: 0008-10-1019 V slot profiles:1 ↔ 0008-10-024 Ranforsare:3
- Mate:126: 0008-10-1020 V slot profiles:3 ↔ 0008-10-024 Ranforsare:3
- Flush:106: 0008-10-1019 V slot profiles:1 ↔ 0008-10-024 Ranforsare:3
- Mate:127: 0008-10-1019 V slot profiles:2 ↔ 0008-10-024 Ranforsare:2
- Mate:128: 0008-10-1020 V slot profiles:2 ↔ 0008-10-024 Ranforsare:2
- Flush:107: 0008-10-1020 V slot profiles:2 ↔ 0008-10-024 Ranforsare:2
- Mate:129: 0008-10-1019 V slot profiles:1 ↔ 0008-10-027 Cutie Arduino:1
- Flush:108: 0008-10-1019 V slot profiles:1 ↔ 0008-10-027 Cutie Arduino:1
- Mate:130: 0008-10-022 Tabla suport:1 ↔ 0008-10-028 Cutie Elemente incalzire:1
- Angle:17 (0 deg): 0008-10-1018 V slot profiles:1 ↔ 0008-10-028 Cutie Elemente incalzire:1
- Mate:131: 0008-10-1020 V slot profiles:2 ↔ 0008-10-024 Ranforsare:4
- Flush:109: 0008-10-1020 V slot profiles:2 ↔ 0008-10-024 Ranforsare:4
- Mate:132: 0008-10-1019 V slot profiles:2 ↔ 0008-10-024 Ranforsare:4
- Insert:12: 0008-10-027 Cutie Arduino:1 ↔ 0008-20-01 Assembly Arduino Mega RAMPS 1.4:1
- Angle:18 (0 deg): 0008-10-027 Cutie Arduino:1 ↔ 0008-20-01 Assembly Arduino Mega RAMPS 1.4:1
- Insert:13: 0008-10-028 Cutie Elemente incalzire:1 ↔ 0008-20-1005 MOSFET_Step:1
- Mate:133: 0008-10-028 Cutie Elemente incalzire:1 ↔ 0008-20-1005 MOSFET_Step:1
- Insert:14: 0008-10-028 Cutie Elemente incalzire:1 ↔ 0008-20-1005 MOSFET_Step:2
- Mate:134: 0008-10-028 Cutie Elemente incalzire:1 ↔ 0008-20-1005 MOSFET_Step:2
- Mate:135: 0008-10-020 Suport Axa Y:4 ↔ 0008-10-028 Cutie Elemente incalzire:1
- Mate:136 (80 mm): 0008-10-1018 V slot profiles:1 ↔ 0008-10-028 Cutie Elemente incalzire:1
- Flush:110 (100 mm): 0008-10-1018 V slot profiles:1 ↔ 0008-10-027 Cutie Arduino:1
- Mate:141: 0008-10-1019 V slot profiles:2 ↔ 0008-10-030 Suport L:4
- Mate:142: 0008-10-1020 V slot profiles:2 ↔ 0008-10-030 Suport L:4
- Flush:113: 0008-10-1019 V slot profiles:2 ↔ 0008-10-030 Suport L:4
- Mate:143: 0008-10-1019 V slot profiles:2 ↔ 0008-10-031 Suport L + placa:1
- Mate:144: 0008-10-1020 V slot profiles:2 ↔ 0008-10-031 Suport L + placa:1
- Flush:114: 0008-10-1019 V slot profiles:2 ↔ 0008-10-031 Suport L + placa:1
- Mate:145: 0008-10-022 Tabla suport:1 ↔ 0008-10-030 Suport L:5
- Mate:146: 0008-10-1019 V slot profiles:2 ↔ 0008-10-030 Suport L:5
- Mate:147: 0008-10-1021  V slot profiles:2 ↔ 0008-10-030 Suport L:5
- Mate:148: 0008-10-022 Tabla suport:1 ↔ 0008-10-030 Suport L:6
- Mate:149: 0008-10-1019 V slot profiles:2 ↔ 0008-10-030 Suport L:6
- Mate:150: 0008-10-1021  V slot profiles:2 ↔ 0008-10-030 Suport L:6
- Mate:151: 0008-10-022 Tabla suport:1 ↔ 0008-10-030 Suport L:7
- Mate:152: 0008-10-1019 V slot profiles:1 ↔ 0008-10-030 Suport L:7
- Mate:153: 0008-10-1021  V slot profiles:1 ↔ 0008-10-030 Suport L:7
- Mate:154: 0008-10-022 Tabla suport:1 ↔ 0008-10-030 Suport L:8
- Mate:155: 0008-10-1021  V slot profiles:1 ↔ 0008-10-030 Suport L:8
- Mate:156: 0008-10-1019 V slot profiles:1 ↔ 0008-10-030 Suport L:8
- Mate:157: 0008-10-1019 V slot profiles:1 ↔ 0008-10-031 Suport L + placa:2
- Mate:158: 0008-10-1020 V slot profiles:3 ↔ 0008-10-031 Suport L + placa:2
- Mate:159: 0008-10-1020 V slot profiles:3 ↔ 0008-10-031 Suport L + placa:2
- Insert:15: 0008-10-1010 Bara 10.ipt:31 ↔ 0008-10-1022 SHF10:4
- Insert:16: 0008-10-1010 Bara 10.ipt:31 ↔ 0008-10-1022 SHF10:1
- Insert:17: 0008-10-1010 Bara 10.ipt:32 ↔ 0008-10-1022 SHF10:3
- Insert:18: 0008-10-1010 Bara 10.ipt:32 ↔ 0008-10-1022 SHF10:2
- Mate:160: 0008-10-022 Tabla suport:1 ↔ 0008-10-1022 SHF10:1
- Angle:19 (0 deg): 0008-10-1019 V slot profiles:2 ↔ 0008-10-1022 SHF10:2
- Angle:20 (0 deg): 0008-10-1019 V slot profiles:1 ↔ 0008-10-1022 SHF10:1
- Mate:161: 0008-10-1018 V slot profiles:3 ↔ 0008-10-032 Suport cadru si axa Z:1
- Mate:162 (0.15 mm): 0008-10-1020 V slot profiles:3 ↔ 0008-10-032 Suport cadru si axa Z:1
- Flush:115: 0008-10-1020 V slot profiles:3 ↔ 0008-10-032 Suport cadru si axa Z:1
- Mate:163: 0008-10-009 X Axis suport.ipt:11 ↔ 0008-10-1010 Bara 10.ipt:31
- Mate:164: 0008-10-009 X Axis suport.ipt:11 ↔ 0008-10-1013 LMK 10 Bearing.ipt:19
- Angle:22 (0 deg): 0008-10-1018 V slot profiles:3 ↔ 0008-10-1022 SHF10:3
- Mate:165: 0008-10-1018 V slot profiles:3 ↔ 0008-10-033:1
- Flush:116: 0008-10-1018 V slot profiles:3 ↔ 0008-10-033:1
- Mate:166: 0008-10-1020 V slot profiles:3 ↔ 0008-10-033:1
- Angle:23 (0 deg): 0008-10-1022 SHF10:4 ↔ 0008-10-033:1
- [Insert]: 0008-10-034 Suport_Rulment:1 ↔ ISO 1224-1 (Metric) 10 - 8 x 16 x 7:3
- Mate:167: 0008-10-033:1 ↔ 0008-10-034 Suport_Rulment:1
- Mate:168: 0008-10-1014 T8 screw.ipt:37 ↔ ISO 1224-1 (Metric) 10 - 8 x 16 x 7:3
- Angle:24 (180 deg): 0008-10-1018 V slot profiles:3 ↔ 0008-10-034 Suport_Rulment:1
- Mate:169: 0008-10-1020 V slot profiles:2 ↔ 0008-10-035:1
- Flush:117: 0008-10-1020 V slot profiles:2 ↔ 0008-10-035:1
- Mate:170: 0008-10-1018 V slot profiles:3 ↔ 0008-10-035:1
- [Insert]: 0008-10-034 Suport_Rulment:2 ↔ ISO 1224-1 (Metric) 10 - 8 x 16 x 7:4
- Mate:171: 0008-10-1014 T8 screw.ipt:38 ↔ 0008-10-035:1
- Insert:21: 0008-10-008 X Axis suport.ipt:12 ↔ 0008-10-013 Supăort Piulita Axa Z.ipt:35
- Mate:172: 0008-10-008 X Axis suport.ipt:12 ↔ 0008-10-013 Supăort Piulita Axa Z.ipt:35
- Mate:173: 0008-10-013 Supăort Piulita Axa Z.ipt:35 ↔ 0008-10-1004 Piulita.ipt:36
- Mate:174: 0008-10-013 Supăort Piulita Axa Z.ipt:35 ↔ 0008-10-1004 Piulita.ipt:36
- Angle:25 (0 deg): 0008-10-008 X Axis suport.ipt:12 ↔ 0008-10-1013 LMK 10 Bearing.ipt:21
- Mate:175: 0008-10-035:1 ↔ 0008-10-034 Suport_Rulment:2
- Mate:176: 0008-10-1014 T8 screw.ipt:38 ↔ ISO 1224-1 (Metric) 10 - 8 x 16 x 7:4
- Mate:177: 0008-10-1018 V slot profiles:3 ↔ 0008-10-032 Suport cadru si axa Z:2
- Flush:118: 0008-10-1020 V slot profiles:2 ↔ 0008-10-032 Suport cadru si axa Z:2
- Mate:178: 0008-10-1020 V slot profiles:2 ↔ 0008-10-032 Suport cadru si axa Z:2
- Insert:22 (0.8 mm): 0008-10-036:1 ↔ 0008-10-1012 16T W6 B3 Without T_Shrinkwrap_1:2
- Flush:120: 0008-10-1011 GT2 Timing Pulley 20 Tooth:4 ↔ 0008-10-1012 16T W6 B3 Without T_Shrinkwrap_1:2
- Angle:27 (0 deg): 0008-10-019 Suport Axa Y:2 ↔ 0008-10-036:1
- Mate:180: 0008-10-022 Tabla suport:1 ↔ 0008-10-037:1
- Mate:181 (0.5 mm): 0008-10-037:1 ↔ 0008-10-036:1
- Mate:182: 0008-10-019 Suport Axa Y:2 ↔ 0008-10-037:1
- Mate:183: 0008-10-1018 V slot profiles:1 ↔ 0008-10-037:1
- Mate:184 (0.5 mm): 0008-10-037:1 ↔ 0008-10-036:1
- Flush:121 (10 mm): 0008-10-1009 LM10uu.ipt:5 ↔ 0008-10-007 Contra suport injectomat.ipt:8
- Flush:122 (20 mm): 0008-10-007 Contra suport injectomat.ipt:8 ↔ 0008-10-1009 LM10uu.ipt:14
- Insert:23: 0008-10-11 ansamblu display:1 ↔ 0008-10-045:1
- Mate:185: 0008-10-11 ansamblu display:1 ↔ 0008-10-045:1
- Insert:24: 0008-10-045:1 ↔ 0008-10-044:1
- Mate:186: 0008-10-1018 V slot profiles:1 ↔ 0008-10-043:1
- Flush:123: 0008-10-1018 V slot profiles:1 ↔ 0008-10-043:1
- Insert:25: 0008-10-044:1 ↔ 0008-10-043:1
- Flush:124 (60 mm): 0008-10-1018 V slot profiles:1 ↔ 0008-10-043:1
- Mate:187: 0008-10-007 Contra suport injectomat.ipt:8 ↔ 0008-20-1003 Switch:1
- Flush:125: 0008-10-007 Contra suport injectomat.ipt:8 ↔ 0008-20-1003 Switch:1
- Flush:126: 0008-10-007 Contra suport injectomat.ipt:8 ↔ 0008-20-1003 Switch:1
- Mate:188: 0008-10-1008 Bara 10_V1.ipt:10 ↔ 0008-10-010 Fixare AxaX:2
- Angle:28 (0 deg): 0008-10-009 X Axis suport.ipt:11 ↔ 0008-10-010 Fixare AxaX:2
- Flush:127: 0008-10-009 X Axis suport.ipt:11 ↔ 0008-10-010 Fixare AxaX:2
- Mate:189: 0008-10-1008 Bara 10_V1.ipt:10 ↔ 0008-10-010 Fixare AxaX:4
- Mate:190 (10 mm): 0008-10-010 Fixare AxaX:2 ↔ 0008-10-010 Fixare AxaX:4
- Mate:191: 0008-10-1008 Bara 10_V1.ipt:10 ↔ 0008-10-010 Fixare AxaX:5
- Angle:29 (0 deg): 0008-10-008 X Axis suport.ipt:12 ↔ 0008-10-010 Fixare AxaX:5
- Flush:128: 0008-10-008 X Axis suport.ipt:12 ↔ 0008-10-010 Fixare AxaX:5
- Mate:192: 0008-10-1008 Bara 10_V1.ipt:10 ↔ 0008-10-010 Fixare AxaX:3
- Flush:129: 0008-10-010 Fixare AxaX:5 ↔ 0008-10-010 Fixare AxaX:3
- Mate:193 (10 mm): 0008-10-010 Fixare AxaX:5 ↔ 0008-10-010 Fixare AxaX:3
- Mate:194: 0008-10-022 Tabla suport:1 ↔ 00008-20-1004 PowerSupplyLedMax500:2
- Flush:130: 00008-20-1004 PowerSupplyLedMax500:1 ↔ 00008-20-1004 PowerSupplyLedMax500:2
- Mate:195: 00008-20-1004 PowerSupplyLedMax500:1 ↔ 00008-20-1004 PowerSupplyLedMax500:2
- Mate:196 (20 mm): 00008-20-1004 PowerSupplyLedMax500:1 ↔ 0008-10-023 Suport L:3
- Mate:197: 0008-10-018 Suport Heated Bed.ipt:52 ↔ 0008-10-047 Suport Rulment Sc si curea:1
- Mate:198: 0008-10-1016 SC10UU:5 ↔ 0008-10-047 Suport Rulment Sc si curea:1
- Mate:199: 0008-10-1016 SC10UU:5 ↔ 0008-10-047 Suport Rulment Sc si curea:1
- Mate:200: 0008-10-1018 V slot profiles:2 ↔ 0008-10-048:1
- Mate:201: 0008-10-1001 NEMA17 - Motor de passo:4 ↔ 0008-10-048:1
- Flush:131: 0008-10-1018 V slot profiles:2 ↔ 0008-10-048:1
- Flush:132: 0008-10-1021  V slot profiles:1 ↔ 0008-10-1021  V slot profiles:2
- Mate:202: 0008-10-015 roata condusa GT2.ipt:41 ↔ 0008-10-1015 Synchronous Belt2.ipt:44
- Insert:26: 0008-10-027 Cutie Arduino:1 ↔ 0008-10-029 Capac Arduino:1
- Angle:30 (0 deg): 0008-10-027 Cutie Arduino:1 ↔ 0008-10-029 Capac Arduino:1
- Mate:203: 0008-10-028 Cutie Elemente incalzire:1 ↔ 0008-10-049 Capac Mofset:1
- Mate:204: 0008-10-028 Cutie Elemente incalzire:1 ↔ 0008-10-049 Capac Mofset:1
- Angle:31 (0 deg): 0008-10-028 Cutie Elemente incalzire:1 ↔ 0008-10-049 Capac Mofset:1
- Mate:205: 0008-10-1019 V slot profiles:1 ↔ Ansamblu nconector priza:1
- Flush:133: 0008-10-1019 V slot profiles:1 ↔ Ansamblu nconector priza:1
- Flush:134: 0008-10-1018 V slot profiles:2 ↔ Ansamblu nconector priza:1
- Mate:206: 0008-20-1003 Switch:2 ↔ 0008-10-056:1
- Flush:135: 0008-20-1003 Switch:2 ↔ 0008-10-056:1
- Flush:136: 0008-20-1003 Switch:2 ↔ 0008-10-056:1
- Mate:207: 0008-10-1020 V slot profiles:3 ↔ 0008-10-056:1
- Flush:137: 0008-10-1020 V slot profiles:3 ↔ 0008-10-056:1
- Mate:208: 0008-10-019 Suport Axa Y.ipt:61 ↔ 0008-20-1003 Switch:3
- Flush:138 (5 mm): 0008-10-019 Suport Axa Y.ipt:61 ↔ 0008-20-1003 Switch:3
- Insert:27: 0008-10-027 Cutie Arduino:1 ↔ 0008-10-026 Suport cutie:1
- Mate:209: 0008-10-027 Cutie Arduino:1 ↔ 0008-10-026 Suport cutie:1
- Insert:28: 0008-10-022 Tabla suport:1 ↔ 0008-10-053 picior:1
- Insert:29: 0008-10-022 Tabla suport:1 ↔ 0008-10-053 picior:5
- Insert:30: 0008-10-022 Tabla suport:1 ↔ 0008-10-053 picior:4
- Insert:31: 0008-10-022 Tabla suport:1 ↔ 0008-10-053 picior:3
- Insert:32: 0008-10-018 Suport Heated Bed.ipt:52 ↔ 0008-10-054 Suport doking:1
- Mate:210: 0008-10-018 Suport Heated Bed.ipt:52 ↔ 0008-10-054 Suport doking:1
- Insert:33: 0008-10-018 Suport Heated Bed.ipt:52 ↔ DIN 7991 M4x20:1
- Insert:34: DIN 315 M4:1 ↔ DIN 7991 M4x20:1
- [Insert]: DIN 315 M4:2 ↔ DIN 7991 M4x20:2
- Insert:36: 0008-10-018 Suport Heated Bed.ipt:52 ↔ DIN 7991 M4x20:2
- Flush:139: 0008-10-054 Suport doking:1 ↔ 0008-10-055 Doking:1
- Angle:32 (0 deg): 0008-10-018 Suport Heated Bed.ipt:52 ↔ 0008-10-055 Doking:1
- Mate:211: 0008-10-054 Suport doking:1 ↔ 0008-10-055 Doking:1
- Mate:212: 0008-10-054 Suport doking:1 ↔ 0008-10-055 Doking:1
- Insert:39: 0008-10-054 Suport doking:1 ↔ DIN 6912 M4 x 25:1
- Insert:40 (-3 mm): DIN 315 M4:3 ↔ DIN 6912 M4 x 25:1
## Named parameters: d120_d113 = 0 mm, d121_d114 = 0 mm, d123_d117 = 0 mm, d124_d118 = 1.5 mm, d125_d119 = 0 mm, d126_d110 = 0 mm, d168_d159 = 0 mm, d169_d160 = 0 mm, d170_d163 = 0 deg, d171_d164 = 0 mm, d172_d165 = 0 mm, d223_d120_d113 = 0 mm, d349_d82 = 0 mm, d358_d349_d82 = 0 mm, d462_d461 = 0 mm
